# Autodesk Inventor assembly: PiZeroAndCameraCases
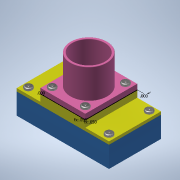
[picture p0: Inventor's stored thumbnail of the model, 180x180]
Saved by Autodesk Inventor 2021 (Build 250183000, 183)
## iProperties
Created: 2018-12-18
Part Number: PiZeroAndCameraCases
Document SubType Name: Assembly
Designer: steele
Author: steele
## Documents named in this file (11)
- C:\git\CAD-Development\robSteele\ShapeWays\TelescopeProjects\PiZeroWCamera\PiZeroAndCameraCases.iam
- C:\git\CAD-Development\robSteele\ShapeWays\TelescopeProjects\PiZeroWCamera\CaseBottomForPiZeroW.ipt
- C:\git\CAD-Development\robSteele\ShapeWays\TelescopeProjects\PiZeroWCamera\CaseTopForPiZeroWandCamera.ipt
- c:\git\CAD-MfgResources\ThingiVerse\Raspberry_Pi_Camera_Module_v2.1_Model\files\RPi_Camera_Module_v2.iam
- C:\git\CAD-Development\robSteele\ShapeWays\TelescopeProjects\PiZeroWCamera\TelescopeAttachementForCase.ipt
- C:\git\CAD-Development\robSteele\ShapeWays\TelescopeProjects\PiZeroWCamera\Pi_Zero_W_ThingIVerse.ipt
- C:\git\CAD-Development\robSteele\ShapeWays\TelescopeProjects\PiZeroWCamera\PiZeroWMechanicalLayout.ipt
- C:\git\CAD-Development\robSteele\ShapeWays\TelescopeProjects\PiZeroWCamera\PiZeroAndCameraCases\Design Accelerator\Bolted Connection5.iam
- c:\git\CAD-MfgResources\McMaster-Carr\BrassHeatSetInsertForPlastic\6-32 0_150 94459A280_BRASS HEAT-SET INSERT FOR PLASTIC.ipt
- C:\git\CAD-Development\robSteele\ShapeWays\TelescopeProjects\PiZeroWCamera\PiZeroAndCameraCases\Design Accelerator\Bolted Connection7.iam
- C:\git\CAD-Development\robSteele\ShapeWays\TelescopeProjects\PiZeroWCamera\PiZeroAndCameraCases\Design Accelerator\Bolted Connection9.iam
## Components (13 placed, 8 different names)
1. CaseBottomForPiZeroW:1 — Mate:3, Flush:1, Flush:2, Insert:5, Insert:6, Insert:7, Insert:8, Insert:23, Insert:24, Insert:25, Insert:26
2. CaseTopForPiZeroWandCamera:1 — Mate:3, Flush:1, Flush:2, Insert:9, Insert:10, Mate:21, Flush:3, Flush:4, Mate:46, Mate:47
3. RPi_Camera_Module_v2:1 [sub-assembly] — Insert:9, Insert:10, Mate:48, Mate:49
4. TelescopeAttachementForCase:1 — Mate:21, Flush:3, Flush:4, Mate:44, Mate:45
5. PiZeroWMechanicalLayout:1 — Insert:5, Insert:6
6. Pi_Zero_W_ThingIVerse:2 — Insert:7, Insert:8
7. Bolted Connection:6 [sub-assembly] — Mate:48, Mate:49
8. Bolted Connection:7 [sub-assembly] — Mate:44, Mate:45
9. Bolted Connection:9 [sub-assembly] — Mate:46, Mate:47
10. 6-32 0_150 94459A280_BRASS HEAT-SET INSERT FOR PLASTIC:6 — Insert:23
11. 6-32 0_150 94459A280_BRASS HEAT-SET INSERT FOR PLASTIC:7 — Insert:24
12. 6-32 0_150 94459A280_BRASS HEAT-SET INSERT FOR PLASTIC:8 — Insert:25
13. 6-32 0_150 94459A280_BRASS HEAT-SET INSERT FOR PLASTIC:9 — Insert:26
## Relationships (22: Insert 10, Mate 8, Flush 4)
- Mate:3: CaseBottomForPiZeroW:1 ↔ CaseTopForPiZeroWandCamera:1
- Flush:1: CaseBottomForPiZeroW:1 ↔ CaseTopForPiZeroWandCamera:1
- Flush:2: CaseBottomForPiZeroW:1 ↔ CaseTopForPiZeroWandCamera:1
- Insert:5: CaseBottomForPiZeroW:1 ↔ PiZeroWMechanicalLayout:1
- Insert:6: CaseBottomForPiZeroW:1 ↔ PiZeroWMechanicalLayout:1
- Insert:7: CaseBottomForPiZeroW:1 ↔ Pi_Zero_W_ThingIVerse:2
- Insert:8: CaseBottomForPiZeroW:1 ↔ Pi_Zero_W_ThingIVerse:2
- Insert:9: CaseTopForPiZeroWandCamera:1 ↔ RPi_Camera_Module_v2:1
- Insert:10: CaseTopForPiZeroWandCamera:1 ↔ RPi_Camera_Module_v2:1
- Mate:21: CaseTopForPiZeroWandCamera:1 ↔ TelescopeAttachementForCase:1
- Flush:3: CaseTopForPiZeroWandCamera:1 ↔ TelescopeAttachementForCase:1
- Flush:4: CaseTopForPiZeroWandCamera:1 ↔ TelescopeAttachementForCase:1
- Insert:23: CaseBottomForPiZeroW:1 ↔ 6-32 0_150 94459A280_BRASS HEAT-SET INSERT FOR PLASTIC:6
- Insert:24: CaseBottomForPiZeroW:1 ↔ 6-32 0_150 94459A280_BRASS HEAT-SET INSERT FOR PLASTIC:7
- Insert:25: CaseBottomForPiZeroW:1 ↔ 6-32 0_150 94459A280_BRASS HEAT-SET INSERT FOR PLASTIC:8
- Insert:26: CaseBottomForPiZeroW:1 ↔ 6-32 0_150 94459A280_BRASS HEAT-SET INSERT FOR PLASTIC:9
- Mate:44: TelescopeAttachementForCase:1 ↔ Bolted Connection:7
- Mate:45: TelescopeAttachementForCase:1 ↔ Bolted Connection:7
- Mate:46: CaseTopForPiZeroWandCamera:1 ↔ Bolted Connection:9
- Mate:47: CaseTopForPiZeroWandCamera:1 ↔ Bolted Connection:9
- Mate:48: RPi_Camera_Module_v2:1 ↔ Bolted Connection:6
- Mate:49: RPi_Camera_Module_v2:1 ↔ Bolted Connection:6
